# Autodesk Inventor assembly: Organ Bank Pretty-Convex Assembly
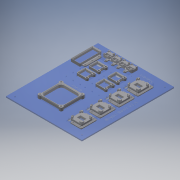
[picture p0: Inventor's stored thumbnail of the model, 180x180]
Saved by Autodesk Inventor 2019 (Build 230136000, 136)
## iProperties
Created: 2021-02-18
Part Number: Organ Bank Pretty-Convex Assembly
Document SubType Name: Assembly
Designer: Eric
Author: Eric
## Documents named in this file (8)
- C:\Users\Eric\Documents\! - Uni\Year 4\MENG PROJECT\Models\My Inventor Models\Designs\Organ Bank Pretty-Convex Assembly.iam
- C:\Users\Eric\Documents\! - Uni\Year 4\MENG PROJECT\Models\My Inventor Models\Designs\Convex Organ Bank Plate.ipt
- C:\Users\Eric\Documents\! - Uni\Year 4\MENG PROJECT\Models\My Inventor Models\Designs\Convex Organ Bank Brain Slot.ipt
- C:\Users\Eric\Documents\! - Uni\Year 4\MENG PROJECT\Models\My Inventor Models\Designs\Convex Organ Bank Castor Slots.ipt
- C:\Users\Eric\Documents\! - Uni\Year 4\MENG PROJECT\Models\My Inventor Models\Designs\Convex Organ Bank Joint Slot.ipt
- C:\Users\Eric\Documents\! - Uni\Year 4\MENG PROJECT\Models\My Inventor Models\Designs\Convex Organ Bank Motor Slot.ipt
- C:\Users\Eric\Documents\! - Uni\Year 4\MENG PROJECT\Models\My Inventor Models\Designs\Convex Organ Bank Sensor Slot.ipt
- C:\Users\Eric\Documents\! - Uni\Year 4\MENG PROJECT\Models\Organ Bank\Eric's Organ Bank.iam
## Components (13 placed, 7 different names)
1. Convex Organ Bank Plate:1 — Flush:1, Flush:2, Flush:3, Mate:2, Mate:3, Flush:8, Flush:9, Mate:6, Mate:10, Mate:11, Mate:12
2. Convex Organ Bank Brain Slot:1 — Mate:1, Tangent:1, Tangent:2, Tangent:3
3. Convex Organ Bank Castor Slots:1 — Mate:2, Flush:4, Flush:5
4. Convex Organ Bank Joint Slot:1 — Flush:6, Flush:7, Mate:3
5. Convex Organ Bank Motor Slot:1 — Mate:8, Flush:10, Flush:13
6. Convex Organ Bank Sensor Slot:1 — Mate:10, Flush:19, Tangent:5
7. Convex Organ Bank Motor Slot:2 — Mate:4, Flush:12, Flush:15
8. Convex Organ Bank Motor Slot:3 — Mate:6, Flush:16, Flush:17
9. Convex Organ Bank Motor Slot:4 — Mate:7, Flush:11, Flush:14
10. Convex Organ Bank Sensor Slot:2 — Mate:11, Flush:20, Tangent:6
11. Convex Organ Bank Sensor Slot:3 — Mate:9, Flush:18, Tangent:4
12. Convex Organ Bank Sensor Slot:4 — Mate:12, Flush:21, Tangent:7
13. Eric's Organ Bank:1 [sub-assembly] — Flush:1, Flush:2, Flush:3, Mate:1, Tangent:1, Tangent:2, Flush:4, Flush:5, Flush:6, Flush:7, Mate:4, Mate:5, Tangent:3, Mate:7, Mate:8, Mate:9, Flush:10, Flush:11, Flush:12, Flush:13, Flush:14, Flush:15, Flush:16, Flush:17, Flush:18, Flush:19, Flush:20, Flush:21, Tangent:4, Tangent:5, Tangent:6, Tangent:7
## Relationships (40: Flush 21, Mate 12, Tangent 7)
- Flush:1: Convex Organ Bank Plate:1 ↔ Eric's Organ Bank:1
- Flush:2: Convex Organ Bank Plate:1 ↔ Eric's Organ Bank:1
- Flush:3: Convex Organ Bank Plate:1 ↔ Eric's Organ Bank:1
- Mate:1: Convex Organ Bank Brain Slot:1 ↔ Eric's Organ Bank:1
- Tangent:1: Convex Organ Bank Brain Slot:1 ↔ Eric's Organ Bank:1
- Tangent:2: Convex Organ Bank Brain Slot:1 ↔ Eric's Organ Bank:1
- Mate:2: Convex Organ Bank Plate:1 ↔ Convex Organ Bank Castor Slots:1
- Flush:4: Convex Organ Bank Castor Slots:1 ↔ Eric's Organ Bank:1
- Flush:5: Convex Organ Bank Castor Slots:1 ↔ Eric's Organ Bank:1
- Flush:6: Convex Organ Bank Joint Slot:1 ↔ Eric's Organ Bank:1
- Flush:7: Convex Organ Bank Joint Slot:1 ↔ Eric's Organ Bank:1
- Mate:3: Convex Organ Bank Plate:1 ↔ Convex Organ Bank Joint Slot:1
- Mate:4: Convex Organ Bank Motor Slot:2 ↔ Eric's Organ Bank:1
- Mate:5: Eric's Organ Bank:1
- Flush:8: Convex Organ Bank Plate:1
- Flush:9: Convex Organ Bank Plate:1
- Tangent:3: Convex Organ Bank Brain Slot:1 ↔ Eric's Organ Bank:1
- Mate:6: Convex Organ Bank Plate:1 ↔ Convex Organ Bank Motor Slot:3
- Mate:7: Convex Organ Bank Motor Slot:4 ↔ Eric's Organ Bank:1
- Mate:8: Convex Organ Bank Motor Slot:1 ↔ Eric's Organ Bank:1
- Mate:9: Convex Organ Bank Sensor Slot:3 ↔ Eric's Organ Bank:1
- Mate:10: Convex Organ Bank Plate:1 ↔ Convex Organ Bank Sensor Slot:1
- Mate:11: Convex Organ Bank Plate:1 ↔ Convex Organ Bank Sensor Slot:2
- Mate:12: Convex Organ Bank Plate:1 ↔ Convex Organ Bank Sensor Slot:4
- Flush:10: Convex Organ Bank Motor Slot:1 ↔ Eric's Organ Bank:1
- Flush:11: Convex Organ Bank Motor Slot:4 ↔ Eric's Organ Bank:1
- Flush:12: Convex Organ Bank Motor Slot:2 ↔ Eric's Organ Bank:1
- Flush:13: Convex Organ Bank Motor Slot:1 ↔ Eric's Organ Bank:1
- Flush:14: Convex Organ Bank Motor Slot:4 ↔ Eric's Organ Bank:1
- Flush:15: Convex Organ Bank Motor Slot:2 ↔ Eric's Organ Bank:1
- Flush:16: Convex Organ Bank Motor Slot:3 ↔ Eric's Organ Bank:1
- Flush:17: Convex Organ Bank Motor Slot:3 ↔ Eric's Organ Bank:1
- Flush:18: Convex Organ Bank Sensor Slot:3 ↔ Eric's Organ Bank:1
- Flush:19: Convex Organ Bank Sensor Slot:1 ↔ Eric's Organ Bank:1
- Flush:20: Convex Organ Bank Sensor Slot:2 ↔ Eric's Organ Bank:1
- Flush:21: Convex Organ Bank Sensor Slot:4 ↔ Eric's Organ Bank:1
- Tangent:4: Convex Organ Bank Sensor Slot:3 ↔ Eric's Organ Bank:1
- Tangent:5: Convex Organ Bank Sensor Slot:1 ↔ Eric's Organ Bank:1
- Tangent:6: Convex Organ Bank Sensor Slot:2 ↔ Eric's Organ Bank:1
- Tangent:7: Convex Organ Bank Sensor Slot:4 ↔ Eric's Organ Bank:1
